# Autodesk Inventor assembly: Hand
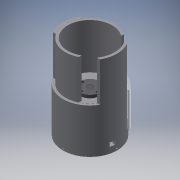
[picture p0: Inventor's stored thumbnail of the model, 180x180]
Saved by Autodesk Inventor 2016 (Build 200138000, 138)
## iProperties
Created: 2016-11-10
Part Number: Hand
Material: 一般
Document SubType Name: Assembly
Designer: Daisuke
Author: Daisuke
## Documents named in this file (6)
- C:\Users\Daisuke\Documents\GitHub\CAD\Hand\ver1\Hand.iam
- C:\Users\Daisuke\Documents\GitHub\CAD\Hand\ver1\insideHand.iam
- C:\Users\Daisuke\Documents\GitHub\CAD\Hand\ver1\outsideHand.iam
- C:\Users\Daisuke\Documents\GitHub\CAD\Hand\ver1\FreeHorn.ipt
- C:\Users\Daisuke\Documents\GitHub\CAD\Hand\ver1\Gear20.ipt
- C:\Users\Daisuke\Documents\GitHub\CAD\Hand\ver1\Servo.ipt
## Components (5 placed, 5 different names)
1. insideHand:1 [sub-assembly] — 挿入:11, 回転:1
2. outsideHand:1 [sub-assembly] — 挿入:8, 挿入:9, 挿入:10, 挿入:11
3. FreeHorn:1 — 挿入:2, 挿入:3, 挿入:4, 挿入:5, 挿入:6, 挿入:7
4. Gear20:1 — 挿入:3, 挿入:4, 挿入:5, 挿入:6, 挿入:7, 回転:1
5. Servo:1 — 挿入:2, 挿入:8, 挿入:9, 挿入:10
## Relationships (11: Insert 10, RelateRotation 1)
- 挿入:2 [Insert]: FreeHorn:1 ↔ Servo:1
- 挿入:3 [Insert]: FreeHorn:1 ↔ Gear20:1
- 挿入:4 [Insert] (1 mm): FreeHorn:1 ↔ Gear20:1
- 挿入:5 [Insert] (1 mm): FreeHorn:1 ↔ Gear20:1
- 挿入:6 [Insert] (1 mm): FreeHorn:1 ↔ Gear20:1
- 挿入:7 [Insert] (1 mm): FreeHorn:1 ↔ Gear20:1
- 挿入:8 [Insert]: outsideHand:1 ↔ Servo:1
- 挿入:9 [Insert]: outsideHand:1 ↔ Servo:1
- 挿入:10 [Insert]: outsideHand:1 ↔ Servo:1
- 挿入:11 [Insert]: insideHand:1 ↔ outsideHand:1
- 回転:1 [RelateRotation] (1 ul): insideHand:1 ↔ Gear20:1
